# Autodesk Inventor assembly: ROBAL_MINI
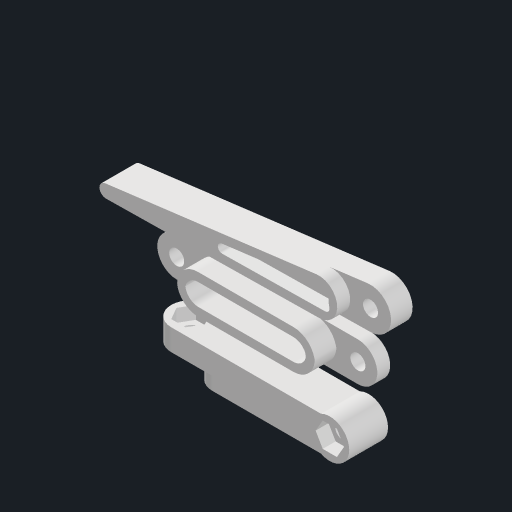
[picture p0: Inventor's stored thumbnail of the model, 512x512]
Saved by Autodesk Inventor 2023.4 (Build 274418000, 418)
## iProperties
Created: 2024-10-16
Part Number: ROBAL_MINI
Document SubType Name: Assembly
Designer: kamil
Author: kamil
## Documents named in this file (4)
- E:\PROJECTS_REPOS\Robal-2.0\mechanics\mini_robal\ROBAL_MINI.iam
- E:\PROJECTS_REPOS\Robal-2.0\mechanics\mini_robal\L3.ipt
- E:\PROJECTS_REPOS\Robal-2.0\mechanics\mini_robal\L2.ipt
- E:\PROJECTS_REPOS\Robal-2.0\mechanics\mini_robal\L1.ipt
## Components (3 placed, 3 different names)
1. L3:1 — Flush:2
2. L2:1 — Flush:1, Flush:2
3. L1:1 — Flush:1
## Relationships (2: Flush 2)
- Flush:1: L2:1 ↔ L1:1
- Flush:2: L3:1 ↔ L2:1
